# Autodesk Inventor assembly: IntakeAssembly.ver-1111-2020
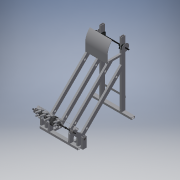
[picture p0: Inventor's stored thumbnail of the model, 180x180]
Saved by Autodesk Inventor 2018 (Build 220112000, 112)
## iProperties
Created: 2020-01-25
Part Number: IntakeAssembly.ver-1111-2020
Document SubType Name: Assembly
Designer: JMHal
Author: JMHal
## Documents named in this file (4)
- E:\PHRC CADD\2020 Infinite Recharge\IntakeAssembly.ver-1111-2020.iam
- E:\PHRC CADD\2020 Infinite Recharge\Intake\Assemblies\IntakeAssembly-ver1-1111-2020.iam
- E:\PHRC CADD\2020 Infinite Recharge\Shooting\Assemblies\ShooterPrototype-ver2-1111-2019.iam
- E:\PHRC CADD\2020 Infinite Recharge\Storage\Assemblies\StorageAssembly.ver4-1111-2020.iam
## Components (3 placed, 3 different names)
1. IntakeAssembly-ver1-1111-2020:1 [sub-assembly]
2. ShooterPrototype-ver2-1111-2019:1 [sub-assembly] — Mate:1, Flush:1, Mate:2
3. StorageAssembly.ver4-1111-2020:1 [sub-assembly] — Mate:1, Flush:1, Mate:2
## Relationships (3: Mate 2, Flush 1)
- Mate:1: ShooterPrototype-ver2-1111-2019:1 ↔ StorageAssembly.ver4-1111-2020:1
- Flush:1: ShooterPrototype-ver2-1111-2019:1 ↔ StorageAssembly.ver4-1111-2020:1
- Mate:2: ShooterPrototype-ver2-1111-2019:1 ↔ StorageAssembly.ver4-1111-2020:1
